# Autodesk Inventor assembly: #SHOOTER.3
(part 2 of 2)
- Mate:166: PURCHASED,BUSHING,13.75mmID,0.75inOD:1 ↔ 3DPRINT,BUSHINGTOHOODDRIVEGEAR,SPACER:1
- Mate:167: 3DPRINT,BUSHINGTOHOODDRIVEGEAR,SPACER:1 ↔ PLATE.HOOD,PINION,GEAR:1
- Mate:168: 3DPRINT,BUSHINGTOHOODDRIVEGEAR,SPACER:2 ↔ STOCK,HEX,ROUND,HOOD:1
- Mate:169: 3DPRINT,BUSHINGTOHOODDRIVEGEAR,SPACER:2 ↔ STOCK,HEX,ROUND,HOOD:1
- Mate:170: PURCHASED,BUSHING,13.75mmID,0.75inOD:2 ↔ 3DPRINT,BUSHINGTOHOODDRIVEGEAR,SPACER:2
- Mate:171: 3DPRINT,SIDEPLATETOHOODGEAR,SPACER:1 ↔ STOCK,HEX,ROUND,HOOD:1
- Mate:172: 3DPRINT,SIDEPLATETOHOODGEAR,SPACER:1 ↔ STOCK,HEX,ROUND,HOOD:1
- Mate:173: PURCHASED,BUSHING,13.75mmID,0.75inOD:1 ↔ 3DPRINT,SIDEPLATETOHOODGEAR,SPACER:1
- Mate:174: PLATE,HOOD,SIDE:1 ↔ PLATE,SHOOTER,BOTTOM:1
- Insert:161: 3DPRINT,HOOD,ALIGNMENT,PLATES:1 ↔ PLATE,HOOD,SIDE:1
- Insert:163: 3DPRINT,HOOD,ALIGNMENT,PLATES:2 ↔ PLATE,HOOD,SIDE:1
- Insert:164: 3DPRINT,HOOD,ALIGNMENT,PLATES:2 ↔ PLATE,HOOD,SIDE:1
- Insert:165: 3DPRINT,HOOD,ALIGNMENT,PLATES:1 ↔ PLATE,HOOD,SIDE:1
- Insert:166: 3DPRINT,HOOD,ALIGNMENT,PLATES:3 ↔ PLATE,HOOD,SIDE:2
- Insert:167: 3DPRINT,HOOD,ALIGNMENT,PLATES:3 ↔ PLATE,HOOD,SIDE:2
- Insert:168: 3DPRINT,HOOD,ALIGNMENT,PLATES:4 ↔ PLATE,HOOD,SIDE:2
- Insert:169: 3DPRINT,HOOD,ALIGNMENT,PLATES:4 ↔ PLATE,HOOD,SIDE:2
- Insert:170: 3DPRINT,HOOD,ALIGNMENT,PLATES:3 ↔ PURCHASED,M3x16mm,BUTTONHEAD,BOLT:1
- Insert:171: 3DPRINT,HOOD,ALIGNMENT,PLATES:3 ↔ PURCHASED,M3x16mm,BUTTONHEAD,BOLT:2
- Insert:172: 3DPRINT,HOOD,ALIGNMENT,PLATES:3 ↔ PURCHASED,M3x16mm,BUTTONHEAD,BOLT:3
- Insert:173: 3DPRINT,HOOD,ALIGNMENT,PLATES:3 ↔ PURCHASED,M3x16mm,BUTTONHEAD,BOLT:4
- Insert:174: 3DPRINT,HOOD,ALIGNMENT,PLATES:1 ↔ PURCHASED,M3x16mm,BUTTONHEAD,BOLT:5
- Insert:175: 3DPRINT,HOOD,ALIGNMENT,PLATES:1 ↔ PURCHASED,M3x16mm,BUTTONHEAD,BOLT:6
- Insert:176: 3DPRINT,HOOD,ALIGNMENT,PLATES:1 ↔ PURCHASED,M3x16mm,BUTTONHEAD,BOLT:7
- Insert:177: 3DPRINT,HOOD,ALIGNMENT,PLATES:1 ↔ PURCHASED,M3x16mm,BUTTONHEAD,BOLT:8
- Insert:178: 3DPRINT,HOOD,ALIGNMENT,PLATES:1 ↔ PURCHASED,M3x16mm,BUTTONHEAD,BOLT:9
- Insert:179: 3DPRINT,HOOD,ALIGNMENT,PLATES:2 ↔ PURCHASED,M3,NYLOCK,NUT:11
- Insert:180: 3DPRINT,HOOD,ALIGNMENT,PLATES:2 ↔ PURCHASED,M3,NYLOCK,NUT:10
- Insert:181: 3DPRINT,HOOD,ALIGNMENT,PLATES:2 ↔ PURCHASED,M3,NYLOCK,NUT:9
- Insert:182: 3DPRINT,HOOD,ALIGNMENT,PLATES:2 ↔ PURCHASED,M3,NYLOCK,NUT:8
- Insert:183: 3DPRINT,HOOD,ALIGNMENT,PLATES:2 ↔ PURCHASED,M3,NYLOCK,NUT:7
- Insert:184: 3DPRINT,HOOD,ALIGNMENT,PLATES:4 ↔ PURCHASED,M3,NYLOCK,NUT:6
- Insert:185: 3DPRINT,HOOD,ALIGNMENT,PLATES:4 ↔ PURCHASED,M3,NYLOCK,NUT:5
- Insert:186: 3DPRINT,HOOD,ALIGNMENT,PLATES:4 ↔ PURCHASED,M3,NYLOCK,NUT:1
- Insert:187: 3DPRINT,HOOD,ALIGNMENT,PLATES:4 ↔ PURCHASED,M3,NYLOCK,NUT:3
- Mate:181 (13.97 mm): PLATE,NUTBLOCK:4 ↔ 3DPRINT,LIMIT_SWITCH,SPACER:1
- Mate:182: 3DPRINT,LIMIT_SWITCH,SPACER:1 ↔ PLATE,SHOOTER,SIDE:1
- Mate:183: 3DPRINT,LIMIT_SWITCH,SPACER:1 ↔ PLATE,SHOOTER,BOTTOM:1
- Mate:184: CONTROLS,LIMIT_SWITCH,VEX:1 ↔ 3DPRINT,LIMIT_SWITCH,SPACER:1
- Mate:185: CONTROLS,LIMIT_SWITCH,VEX:1 ↔ PLATE,SHOOTER,BOTTOM:1
- Mate:186: CONTROLS,LIMIT_SWITCH,VEX:1 ↔ 3DPRINT,LIMIT_SWITCH,SPACER:1
- Mate:187: PURCHASED,M4x12mm,BUTTONHEAD,BOLT:9 ↔ PLATE,SHOOTER,SIDE:1
- Mate:188: CONTROLS,LIMIT_SWITCH,VEX:1 ↔ PURCHASED,M4x12mm,BUTTONHEAD,BOLT:9
- Mate:189: PURCHASED,M4x12mm,BUTTONHEAD,BOLT:10 ↔ PLATE,SHOOTER,SIDE:1
- Mate:190: CONTROLS,LIMIT_SWITCH,VEX:1 ↔ PURCHASED,M4x12mm,BUTTONHEAD,BOLT:10
- Insert:188: CONTROLS,SPARK_FLEX:1 ↔ PLATE,HOOD,SIDE:1
- Insert:191: CONTROLS,SPARK_FLEX:2 ↔ PLATE,HOOD,SIDE:2
- Mate:191: PURCHASED,HEX_BEARING:1 ↔ PURCHASED,WASHER:5
- Mate:192: PURCHASED,HEX_BEARING:1 ↔ 3DPRINT,SIDEPLATETOHOOD,SPACER :2
- Mate:193: PLATE,NUTBLOCK:5 ↔ PLATE,SHOOTER,BOTTOM:1
- Mate:194: PURCHASED,HEX_BEARING:5 ↔ 3DPRINT,BACKROLLERS,OPENSIDE,SPACER:1
- Insert:192: PLATE,SHOOTER,BACK:1 ↔ PLATE,SHOOTER,SIDE:2
- Insert:193: PLATE,SHOOTER,BACK:1 ↔ PLATE,SHOOTER,SIDE:2
- Insert:195: PURCHASED,10-32x0.5in,BUTTONHEAD,BOLT:53 ↔ PLATE,SHOOTER,SIDE:1
- Insert:198: PURCHASED,10-32x0.5in,BUTTONHEAD,BOLT:56 ↔ PLATE,SHOOTER,SIDE:2
- Insert:199: PURCHASED,10-32x0.5in,BUTTONHEAD,BOLT:59 ↔ PLATE,HOOD,SIDE:2
- Insert:200: PURCHASED,10-32x0.5in,BUTTONHEAD,BOLT:58 ↔ PLATE,HOOD,SIDE:2
- Insert:201: PURCHASED,10-32x0.5in,BUTTONHEAD,BOLT:57 ↔ PLATE,HOOD,SIDE:2
- Insert:202: PURCHASED,10-32x0.5in,BUTTONHEAD,BOLT:62 ↔ PLATE,HOOD,SIDE:2
- Insert:203: PURCHASED,10-32x0.5in,BUTTONHEAD,BOLT:60 ↔ PLATE,HOOD,SIDE:2
- Insert:204: PURCHASED,10-32x0.5in,BUTTONHEAD,BOLT:61 ↔ PLATE,HOOD,SIDE:2
- Insert:205: PURCHASED,10-32x0.5in,BUTTONHEAD,BOLT:63 ↔ PLATE,HOOD,SIDE:1
- Insert:206: PURCHASED,10-32x0.5in,BUTTONHEAD,BOLT:66 ↔ PLATE,HOOD,SIDE:1
- Insert:207: PURCHASED,10-32x0.5in,BUTTONHEAD,BOLT:64 ↔ PLATE,HOOD,SIDE:1
- Insert:208: PURCHASED,10-32x0.5in,BUTTONHEAD,BOLT:65 ↔ PLATE,HOOD,SIDE:1
- Insert:209: PURCHASED,10-32x0.5in,BUTTONHEAD,BOLT:68 ↔ PLATE,HOOD,SIDE:1
- Insert:210: PURCHASED,10-32x0.5in,BUTTONHEAD,BOLT:67 ↔ PLATE,HOOD,SIDE:1
- Mate:196: 3DPRINT,LIMIT_SWITCH,SPACER,RIGHT:1 ↔ PLATE,SHOOTER,SIDE:2
- Mate:197: 3DPRINT,LIMIT_SWITCH,SPACER,RIGHT:1 ↔ PLATE,SHOOTER,SIDE:2
- Mate:198: CONTROLS,LIMIT_SWITCH,VEX:2 ↔ 3DPRINT,LIMIT_SWITCH,SPACER,RIGHT:1
- Mate:199: CONTROLS,LIMIT_SWITCH,VEX:2 ↔ 3DPRINT,LIMIT_SWITCH,SPACER,RIGHT:1
- Mate:200: CONTROLS,LIMIT_SWITCH,VEX:2 ↔ 3DPRINT,LIMIT_SWITCH,SPACER,RIGHT:1
- Mate:201: PURCHASED,M4x12mm,BUTTONHEAD,BOLT:11 ↔ PLATE,SHOOTER,SIDE:2
- Mate:202: PURCHASED,M4x12mm,BUTTONHEAD,BOLT:12 ↔ PLATE,SHOOTER,SIDE:2
- Mate:203: CONTROLS,LIMIT_SWITCH,VEX:2 ↔ PURCHASED,M4x12mm,BUTTONHEAD,BOLT:12
- Mate:204: CONTROLS,LIMIT_SWITCH,VEX:2 ↔ PURCHASED,M4x12mm,BUTTONHEAD,BOLT:11
- Flush:10: 3DPRINT,LIMIT_SWITCH,SPACER:1 ↔ 3DPRINT,LIMIT_SWITCH,SPACER,RIGHT:1
- Mate:207: PLATE,FLYWHEEL,HUB:1 ↔ STOCK,SHAFT,HEX,SHOOTER:1
- Mate:208: PLATE,FLYWHEEL,HUB:1 ↔ STOCK,SHAFT,HEX,SHOOTER:1
- Mate:209: MOTOR,REV,NEO,VORTEX:2 ↔ PLATE,FLYWHEEL,HUB:1
- Mate:210: PLATE,SHOOTER,BOTTOM:1
- Mate:211: PLATE,SHOOTER,BOTTOM:1
- Mate:212: 3DPRINT,BACKRAIL:1 ↔ PURCHASED,M4x12mm,BUTTONHEAD,BOLT:2
- Rotation:1 [RelateRotation] (1 ul): STOCK,SHAFT,HEX,HOOD,WHEELS,LONG:1 ↔ STOCK,SHAFT,HEX,HOOD,REVERSER:1
- Rotation:2 [RelateRotation] (1 ul): STOCK,SHAFT,HEX,HOOD,WHEELS,LONG:1 ↔ STOCK,SHAFT,HEX,HOOD,REVERSER:1
- Rotation:3 [RelateRotation] (1 ul): STOCK,SHAFT,HEX,HOOD,WHEELS,LONG:1 ↔ STOCK,SHAFT,HEX,HOOD,WHEELS,SHORT:1
- Rotation:4 [RelateRotation] (1 ul): STOCK,SHAFT,HEX,SHOOTER:1 ↔ STOCK,SHAFT,HEX,HOOD,REVERSER:1
- Mate:214: PLATE,FLYWHEEL,HUB:1 ↔ CAST,FLYWHEEL,GRIP:2
- Flush:12: PLATE,FLYWHEEL,HUB:1 ↔ CAST,FLYWHEEL,GRIP:2
- Mate:215: PLATE,FLYWHEEL,HUB:1 ↔ CAST,FLYWHEEL,GRIP:2
- Mate:216: CONTROLS,SPARK_MAX:1 ↔ PLATE,SHOOTER,BACK:1
- Mate:217: 3DPRINT,SPARK_MAX,MOUNT:1 ↔ PLATE,SHOOTER,BACK:1
- Mate:218: 3DPRINT,SPARK_MAX,MOUNT:1 ↔ PLATE,SHOOTER,BACK:1
- Mate:220: CONTROLS,SPARK_MAX:1 ↔ 3DPRINT,SPARK_MAX,MOUNT:1
- Mate:221: CONTROLS,SPARK_MAX:1 ↔ 3DPRINT,SPARK_MAX,MOUNT:1
- Insert:219: CONTROLS,SPARK_FLEX:1 ↔ PLATE,HOOD,SIDE:1
- Insert:220: CONTROLS,SPARK_FLEX:2 ↔ PLATE,HOOD,SIDE:2
- Mate:224: 3DPRINT,SPARK_MAX,MOUNT:1 ↔ PLATE,SHOOTER,BACK:1
- Mate:225: 3DPRINT,BACKRAIL:1 ↔ PLATE,SHOOTER,BOTTOM:1
- Insert:221: PURCHASED,10-32x0.625in,FLATHEAD,BOLT:1 ↔ PLATE,SHOOTER,BOTTOM:1
- Insert:222: PURCHASED,10-32x0.5in,BUTTONHEAD,BOLT:69 ↔ PLATE,SHOOTER,BOTTOM:1
- Insert:223: PURCHASED,10-32x0.5in,BUTTONHEAD,BOLT:70 ↔ PLATE,SHOOTER,BOTTOM:1
- Insert:224: PURCHASED,10-32x0.5in,BUTTONHEAD,BOLT:71 ↔ PLATE,SHOOTER,BOTTOM:1
- Insert:225: PURCHASED,10-32x0.5in,BUTTONHEAD,BOLT:72 ↔ PLATE,SHOOTER,BOTTOM:1
- Insert:226: PURCHASED,10-32x0.5in,BUTTONHEAD,BOLT:73 ↔ PLATE,SHOOTER,BOTTOM:1
- Insert:227: PURCHASED,10-32x0.5in,BUTTONHEAD,BOLT:74 ↔ PLATE,SHOOTER,BOTTOM:1
- Insert:228: PURCHASED,10-32x0.5in,BUTTONHEAD,BOLT:75 ↔ PLATE,SHOOTER,BOTTOM:1
- Insert:229: PURCHASED,10-32x0.5in,BUTTONHEAD,BOLT:76 ↔ PLATE,SHOOTER,SIDE:1
- Insert:230: PURCHASED,10-32x0.5in,BUTTONHEAD,BOLT:77 ↔ PLATE,SHOOTER,SIDE:2
- Mate:226: PURCHASED,HEX_BEARING:15 ↔ 3DPRINT,REVERSERGEAR,SPACER,SHORT:1
- Mate:227: PURCHASED,HTD5mm,20T,PULLEY:4 ↔ 3DPRINT,REVERSERGEAR,SPACER,SHORT:1
- Mate:228: 3DPRINT,CABLE,GUARD:1 ↔ 3DPRINT,CABLE,GUARD:2
- Mate:229: 3DPRINT,CABLE,GUARD:1 ↔ 3DPRINT,CABLE,GUARD:2
- Mate:230: 3DPRINT,CABLE,GUARD:1 ↔ 3DPRINT,CABLE,GUARD:2
- Mate:231: 3DPRINT,CABLE,GUARD:2 ↔ 3DPRINT,CABLE,GUARD:3
- Mate:232: 3DPRINT,CABLE,GUARD:2 ↔ 3DPRINT,CABLE,GUARD:3
- Mate:233: 3DPRINT,CABLE,GUARD:2 ↔ 3DPRINT,CABLE,GUARD:3
- Mate:234: 3DPRINT,CABLE,GUARD:3 ↔ 3DPRINT,CABLE,GUARD:4
- Mate:235: 3DPRINT,CABLE,GUARD:3 ↔ 3DPRINT,CABLE,GUARD:4
- Mate:236: 3DPRINT,CABLE,GUARD:3 ↔ 3DPRINT,CABLE,GUARD:4
- Mate:237: 3DPRINT,CABLE,GUARD:1 ↔ PLATE,SHOOTER,BOTTOM:1
- Mate:238: 3DPRINT,CABLE,GUARD:1 ↔ PLATE,SHOOTER,BOTTOM:1
- Mate:239: 3DPRINT,CABLE,GUARD:4 ↔ PLATE,SHOOTER,BOTTOM:1
- Insert:231: PURCHASED,HEX_BEARING:12 ↔ PLATE,HOOD,SIDE:2
- Insert:232: PURCHASED,M4x12mm,BUTTONHEAD,BOLT:1 ↔ PLATE,SHOOTER,BOTTOM:1
- Insert:233: PURCHASED,M4x12mm,BUTTONHEAD,BOLT:4 ↔ PLATE,SHOOTER,BOTTOM:1
- Insert:234: PURCHASED,M4x12mm,BUTTONHEAD,BOLT:3 ↔ PLATE,SHOOTER,BOTTOM:1
- Insert:235: PURCHASED,M4x12mm,BUTTONHEAD,BOLT:8 ↔ PLATE,SHOOTER,BOTTOM:1
- Insert:236: PURCHASED,M4x12mm,BUTTONHEAD,BOLT:7 ↔ PLATE,SHOOTER,BOTTOM:1
- Insert:237: PURCHASED,M4x12mm,BUTTONHEAD,BOLT:5 ↔ PLATE,SHOOTER,BOTTOM:1
- Mate:240: 3DPRINT,BACKRAIL_MIR:1 ↔ PLATE,SHOOTER,BOTTOM:1
- Mate:241: 3DPRINT,BACKRAIL_MIR:1 ↔ PLATE,SHOOTER,BOTTOM:1
- Mate:242: 3DPRINT,BACKRAIL_MIR:1 ↔ PLATE,SHOOTER,BOTTOM:1
- Mate:243: PURCHASED,2inOD,HEX,SHOOTER,WHEEL:1 ↔ 3DPRINT,BACKROLLERS,PULLEYSIDE,SPACER:1
- Mate:244: PURCHASED,2inOD,HEX,SHOOTER,WHEEL:3 ↔ 3DPRINT,BACKROLLERS,PULLEYSIDE,SPACER:2
- Mate:245: 3DPRINT,BACKROLLERS,PULLEY,SPACER:1 ↔ STOCK,SHAFT,HEX,HOOD,WHEELS,SHORT:1
- Mate:246: PURCHASED,HTD5mm,20T,PULLEY:2 ↔ 3DPRINT,BACKROLLERS,PULLEY,SPACER:1
- Mate:247: 3DPRINT,BACKROLLERS,PULLEY,SPACER:2 ↔ STOCK,SHAFT,HEX,HOOD,WHEELS,LONG:1
- Mate:248: PURCHASED,HTD5mm,20T,PULLEY:1 ↔ 3DPRINT,BACKROLLERS,PULLEY,SPACER:2
- Mate:249: 3DPRINT,BACKROLLERS,PULLEY,SPACER:2 ↔ STOCK,SHAFT,HEX,HOOD,WHEELS,LONG:1
- Mate:250: 3DPRINT,BACKROLLERS,PULLEY,SPACER:1 ↔ STOCK,SHAFT,HEX,HOOD,WHEELS,SHORT:1
- Insert:238: PLATE,NUTBLOCK,BACK:1 ↔ PLATE,SHOOTER,BACK:1
- Insert:239: PLATE,NUTBLOCK,BACK:1 ↔ PLATE,SHOOTER,BACK:1
- Insert:240: 3DPRINT,SPARK_MAX,MOUNT:1 ↔ PURCHASED,10-32x0.5in,BUTTONHEAD,BOLT:78
- Insert:241: 3DPRINT,SPARK_MAX,MOUNT:1 ↔ PURCHASED,10-32x0.5in,BUTTONHEAD,BOLT:79
- Insert:242: 3DPRINT,SPARK_MAX,MOUNT:1 ↔ PURCHASED,10-32x0.5in,BUTTONHEAD,BOLT:80
- Insert:243: STOCK,ROUND,0.375inOD,10-32,STANDOFF:1 ↔ PLATE,HOOD,SIDE:2
- Insert:244: STOCK,ROUND,0.375inOD,10-32,STANDOFF:2 ↔ PLATE,HOOD,SIDE:2
- Insert:245: STOCK,ROUND,0.375inOD,10-32,STANDOFF:3 ↔ PLATE,HOOD,SIDE:2
